# Autodesk Inventor assembly: 足回り製作中
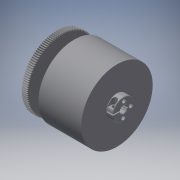
[picture p0: Inventor's stored thumbnail of the model, 180x180]
Saved by Autodesk Inventor 2019 (Build 230136000, 136)
## iProperties
Created: 2020-09-22
Part Number: 足回り製作中
Material: 一般
Document SubType Name: Assembly
Designer: zhept
Author: zhept
## iProperties of the stored document _SCS  1010CP3-part.ipt
Created: 2020-09-22
Part Number: _SCS  1010CP3-part
Material: 一般
Document SubType Name: Modeling
Designer: zhept
Density: 1 g/cm^3
Appearance: 既定
Author: zhept
Revision Number: NONE
## iProperties of the stored document SCS1010CP3.iam
Created: 2020-09-22
Part Number: SCS1010CP3
Material: 一般
Description: STEP AP214
Document SubType Name: Assembly
Designer: zhept
Company: CADENAS
Title: p:/temp/worker_11/temp/exporttempdir_1548_111_LzgDy/format_0/SCS1010CP3.stp
Author: License CC BY-ND 4.0
Revision Number: NONE
Sending System: PARTsolutions
## Documents named in this file (6)
- C:\Users\zhept\OneDrive\大学\rrst\足回り2020\足回り製作中.iam
- **C:\Users\zhept\OneDrive\大学\rrst\足回り2020\足回り製作中.iam*LocalDocs*x5xzzs5k5Jsdvuuwr3r2whv0gVg*SCS1010CP3.iam
- C:\Users\zhept\OneDrive\大学\rrst\ローラー\ローラー.ipt
- C:\Users\zhept\OneDrive\大学\rrst\足回り2020\KHK_SS08120AOn\SS0.8-120A_On.ipt
- C:\Users\zhept\OneDrive\大学\rrst\IWATA_SCS1010CP3\SCS1010CP3.stp
- **C:\Users\zhept\OneDrive\大学\rrst\足回り2020\足回り製作中.iam*LocalDocs*xC2tchb2vJyzuuj0h3sugloszYg*_SCS  1010CP3-part.ipt
## Components (4 placed, 3 different names)
1. SCS1010CP3:1 [sub-assembly] — 挿入:1, 挿入:2, 挿入:4
2. ローラー:1 — 挿入:1, 挿入:2, 挿入:3, メイト:1
3. SCS1010CP3:2 [sub-assembly] — 挿入:3, メイト:1
4. SS0.8-120A_On:1 — 挿入:4
## Relationships (5: Insert 4, Mate 1)
- 挿入:1 [Insert]: SCS1010CP3:1 ↔ ローラー:1
- 挿入:2 [Insert]: SCS1010CP3:1 ↔ ローラー:1
- 挿入:3 [Insert]: ローラー:1 ↔ SCS1010CP3:2
- メイト:1 [Mate]: ローラー:1 ↔ SCS1010CP3:2
- 挿入:4 [Insert]: SCS1010CP3:1 ↔ SS0.8-120A_On:1
